# Autodesk Inventor assembly: Assembly
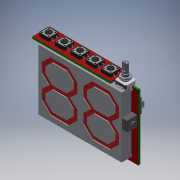
[picture p0: Inventor's stored thumbnail of the model, 180x180]
Saved by Autodesk Inventor 2019.3 (Build 233278000, 278)
## iProperties
Created: 2019-03-27
Part Number: Assembly
Document SubType Name: Assembly
Designer: Willist
Author: Willist
## Documents named in this file (8)
- D:\Biblioteki\Dokumenty\,Studia\Magistarka\Projekt Grupowy\Minutnik\Projekt-Grupowy-Minutnik\CAD\Assembly.iam
- D:\Biblioteki\Dokumenty\,Studia\Magistarka\Projekt Grupowy\Minutnik\Projekt-Grupowy-Minutnik\CAD\Digit.ipt
- D:\Biblioteki\Dokumenty\,Studia\Magistarka\Projekt Grupowy\Minutnik\Projekt-Grupowy-Minutnik\CAD\MainBoard.ipt
- D:\Biblioteki\Dokumenty\,Studia\Magistarka\Projekt Grupowy\Minutnik\Projekt-Grupowy-Minutnik\CAD\R1206.ipt
- D:\Biblioteki\Dokumenty\,Studia\Magistarka\Projekt Grupowy\Minutnik\Projekt-Grupowy-Minutnik\CAD\Charger.ipt
- D:\Biblioteki\Dokumenty\,Studia\Magistarka\Projekt Grupowy\Minutnik\Projekt-Grupowy-Minutnik\CAD\OnOffSwitch.ipt
- D:\Biblioteki\Dokumenty\,Studia\Magistarka\Projekt Grupowy\Minutnik\Projekt-Grupowy-Minutnik\CAD\AssUpper.iam
- D:\Biblioteki\Dokumenty\,Studia\Magistarka\Projekt Grupowy\Minutnik\Projekt-Grupowy-Minutnik\CAD\Encoder incremental.ipt
## Components (8 placed, 7 different names)
1. Digit:1 — Mate:1
2. Digit:2 — Mate:1
3. MainBoard:1
4. R1206:1
5. Charger:1
6. OnOffSwitch:1
7. AssUpper:1 [sub-assembly]
8. Encoder incremental:1
## Relationships (1: Mate 1)
- Mate:1: Digit:1 ↔ Digit:2
